# Autodesk Inventor assembly: B_Legs0
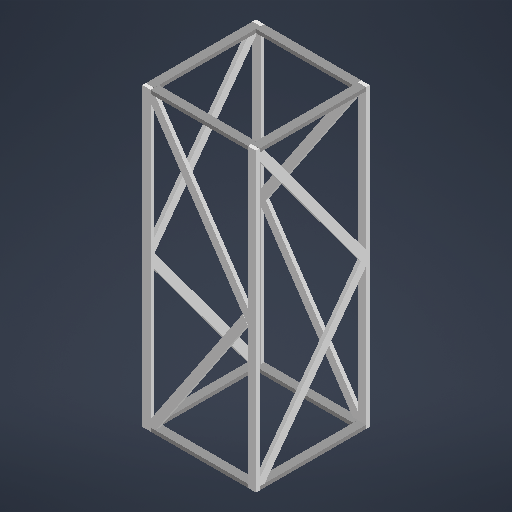
[picture p0: Inventor's stored thumbnail of the model, 512x512]
Saved by Autodesk Inventor 2026 (Build 300175000, 175)
## iProperties
Created: 2024-09-19
Part Number: B_Legs0
Document SubType Name: Assembly
Designer: User
Author: User
## Documents named in this file (8)
- C:\Users\trott\Documents\UofSC-ASME-Tiger-Burn-Design-2025\CAD\Legs\Front Leg\F_Leg.iam
- C:\Users\trott\Documents\UofSC-ASME-Tiger-Burn-Design-2025\CAD\Legs\Front Leg\2x4x41.ipt
- C:\Users\trott\Documents\UofSC-ASME-Tiger-Burn-Design-2025\CAD\Legs\Front Leg\2x4x125.ipt
- C:\Users\trott\Documents\UofSC-ASME-Tiger-Burn-Design-2025\CAD\Legs\Front Leg\S_2x4x76.102.ipt
- C:\Users\trott\Documents\UofSC-ASME-Tiger-Burn-Design-2025\CAD\Legs\Front Leg\S_2x4x73.498.ipt
- C:\Users\trott\Documents\UofSC-ASME-Tiger-Burn-Design-2025\CAD\Legs\Front Leg\2x4x45.ipt
- C:\Users\trott\Documents\UofSC-ASME-Tiger-Burn-Design-2025\CAD\Legs\Front Leg\S_2x4x75.802.ipt
- C:\Users\trott\Documents\UofSC-ASME-Tiger-Burn-Design-2025\CAD\Legs\Front Leg\S_2x4x78.175.ipt
## Components (20 placed, 7 different names)
1. 2x4x41:5 — Flush:27, Mate:18, Flush:28, Mate:34
2. S_2x4x73.498:2 — Mate:33, Mate:34, Flush:48, Mate:53
3. 2x4x45:1 — Mate:35, Flush:49, Mate:37, Mate:39, Flush:52, Mate:58, Mate:60, Mate:61, Mate:72
4. 2x4x41:6 — Mate:38, Flush:50, Flush:51, Mate:41, Flush:67, Mate:55, Mate:57, Mate:58, Mate:59, Mate:64
5. 2x4x41:7 — Mate:39, Flush:52, Flush:53, Mate:52, Mate:60, Mate:62
6. 2x4x45:2 — Mate:40, Flush:54, Mate:41, Mate:56, Mate:57, Mate:70
7. 2x4x45:3 — Mate:42, Flush:55, Flush:56, Mate:66
8. 2x4x45:4 — Mate:43, Flush:57, Flush:58, Flush:59, Flush:60, Mate:68
9. 2x4x41:8 — Mate:44, Flush:61, Flush:62, Mate:46
10. S_2x4x73.498:3 — Mate:45, Flush:63, Mate:46
11. S_2x4x76.102:1 — Mate:51, Mate:52, Flush:66, Mate:53
12. S_2x4x76.102:4 — Mate:63, Mate:64, Flush:68
13. S_2x4x75.802:1 — Mate:65, Flush:69, Mate:66
14. S_2x4x75.802:2 — Mate:67, Mate:68, Flush:70
15. S_2x4x78.175:1 — Mate:69, Mate:70, Flush:71
16. S_2x4x78.175:2 — Mate:71, Mate:72, Flush:72
17. 2x4x125:2 — Mate:40, Flush:54, Mate:43, Flush:59, Flush:60, Mate:45, Flush:63, Flush:67, Mate:55, Mate:56, Mate:63, Flush:68
18. 2x4x125:1 — Flush:27, Mate:18, Flush:28, Flush:57, Flush:58, Mate:67, Flush:70, Mate:69, Flush:71
19. 2x4x125:3 — Mate:35, Flush:49, Mate:38, Flush:50, Flush:51, Mate:42, Mate:44, Flush:61, Flush:62, Mate:59, Mate:65, Flush:69, Mate:71, Flush:72
20. 2x4x125:4 — Mate:33, Flush:48, Mate:37, Flush:53, Flush:55, Flush:56, Mate:51, Flush:66, Mate:61, Mate:62
## Component patterns: (2 elements, first: 2x4x125:2 + 2x4x125:1)
## Relationships (60: Mate 35, Flush 25)
- Flush:27: 2x4x41:5 ↔ 2x4x125:1
- Mate:18: 2x4x41:5 ↔ 2x4x125:1
- Flush:28: 2x4x41:5 ↔ 2x4x125:1
- Mate:33: S_2x4x73.498:2 ↔ 2x4x125:4
- Mate:34: 2x4x41:5 ↔ S_2x4x73.498:2
- Flush:48: S_2x4x73.498:2 ↔ 2x4x125:4
- Mate:35: 2x4x45:1 ↔ 2x4x125:3
- Flush:49: 2x4x45:1 ↔ 2x4x125:3
- Mate:37: 2x4x45:1 ↔ 2x4x125:4
- Mate:38: 2x4x41:6 ↔ 2x4x125:3
- Flush:50: 2x4x41:6 ↔ 2x4x125:3
- Flush:51: 2x4x41:6 ↔ 2x4x125:3
- Mate:39: 2x4x45:1 ↔ 2x4x41:7
- Flush:52: 2x4x45:1 ↔ 2x4x41:7
- Flush:53: 2x4x41:7 ↔ 2x4x125:4
- Mate:40: 2x4x45:2 ↔ 2x4x125:2
- Flush:54: 2x4x45:2 ↔ 2x4x125:2
- Mate:41: 2x4x41:6 ↔ 2x4x45:2
- Mate:42: 2x4x45:3 ↔ 2x4x125:3
- Flush:55: 2x4x45:3 ↔ 2x4x125:4
- Flush:56: 2x4x45:3 ↔ 2x4x125:4
- Mate:43: 2x4x45:4 ↔ 2x4x125:2
- Flush:57: 2x4x45:4 ↔ 2x4x125:1
- Flush:58: 2x4x45:4 ↔ 2x4x125:1
- Flush:59: 2x4x45:4 ↔ 2x4x125:2
- Flush:60: 2x4x45:4 ↔ 2x4x125:2
- Mate:44: 2x4x41:8 ↔ 2x4x125:3
- Flush:61: 2x4x41:8 ↔ 2x4x125:3
- Flush:62: 2x4x41:8 ↔ 2x4x125:3
- Mate:45: S_2x4x73.498:3 ↔ 2x4x125:2
- Flush:63: S_2x4x73.498:3 ↔ 2x4x125:2
- Mate:46: 2x4x41:8 ↔ S_2x4x73.498:3
- Mate:51: S_2x4x76.102:1 ↔ 2x4x125:4
- Mate:52: 2x4x41:7 ↔ S_2x4x76.102:1
- Flush:66: S_2x4x76.102:1 ↔ 2x4x125:4
- Mate:53: S_2x4x73.498:2 ↔ S_2x4x76.102:1
- Flush:67: 2x4x41:6 ↔ 2x4x125:2
- Mate:55: 2x4x41:6 ↔ 2x4x125:2
- Mate:56: 2x4x45:2 ↔ 2x4x125:2
- Mate:57: 2x4x41:6 ↔ 2x4x45:2
- Mate:58: 2x4x45:1 ↔ 2x4x41:6
- Mate:59: 2x4x41:6 ↔ 2x4x125:3
- Mate:60: 2x4x45:1 ↔ 2x4x41:7
- Mate:61: 2x4x45:1 ↔ 2x4x125:4
- Mate:62: 2x4x41:7 ↔ 2x4x125:4
- Mate:63: S_2x4x76.102:4 ↔ 2x4x125:2
- Mate:64: 2x4x41:6 ↔ S_2x4x76.102:4
- Flush:68: S_2x4x76.102:4 ↔ 2x4x125:2
- Mate:65: S_2x4x75.802:1 ↔ 2x4x125:3
- Flush:69: S_2x4x75.802:1 ↔ 2x4x125:3
- Mate:66: 2x4x45:3 ↔ S_2x4x75.802:1
- Mate:67: S_2x4x75.802:2 ↔ 2x4x125:1
- Mate:68: 2x4x45:4 ↔ S_2x4x75.802:2
- Flush:70: S_2x4x75.802:2 ↔ 2x4x125:1
- Mate:69: S_2x4x78.175:1 ↔ 2x4x125:1
- Mate:70: 2x4x45:2 ↔ S_2x4x78.175:1
- Flush:71: S_2x4x78.175:1 ↔ 2x4x125:1
- Mate:71: S_2x4x78.175:2 ↔ 2x4x125:3
- Mate:72: 2x4x45:1 ↔ S_2x4x78.175:2
- Flush:72: S_2x4x78.175:2 ↔ 2x4x125:3
